# Autodesk Inventor assembly: VisiStick Assembly
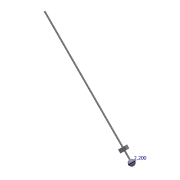
[picture p0: Inventor's stored thumbnail of the model, 180x180]
Saved by Autodesk Inventor 2018.3 (Build 223284000, 284)
## iProperties
Created: 2018-11-06
Part Number: VisiStick Assembly
Document SubType Name: Assembly
Designer: aye06091
Mass: 307.754 g
Surface Area: 719.761 cm^2
Volume: 307.754 cm^3
Density: 1 g/cm^3
Author: aye06091
## Documents named in this file (3)
- \\niskyschools.org\dfs\Student\Home\GY2019\tei06398\VisiStick\VisiStick Assembly.iam
- \\niskyschools.org\dfs\Student\Home\GY2019\tei06398\VisiStick\VisiStick.ipt
- \\niskyschools.org\dfs\Student\Home\GY2019\tei06398\VisiStick\Lidar Holder 1.ipt
## Components (2 placed, 2 different names)
1. VisiStick:1 — Insert:1
2. Lidar Holder 1:1 — Insert:1
## Relationships (1: Insert 1)
- Insert:1 (-127 mm): VisiStick:1 ↔ Lidar Holder 1:1
